# Autodesk Inventor assembly: toe_joint
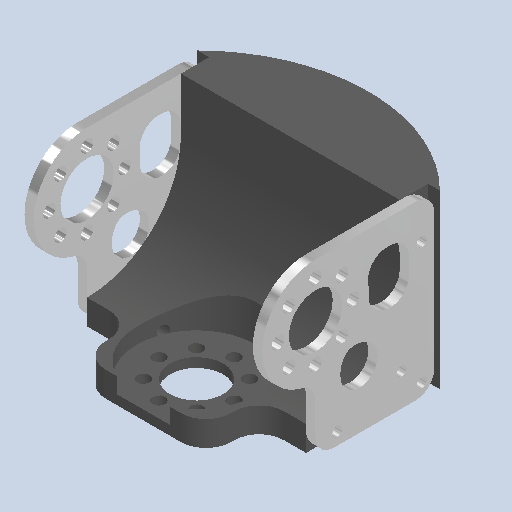
[picture p0: Inventor's stored thumbnail of the model, 512x512]
Saved by Autodesk Inventor 2024.1 (Build 281209000, 209)
## iProperties
Created: 2024-02-11
Part Number: toe_joint
Document SubType Name: Assembly
Designer: hibik
Author: hibik
## Documents named in this file (3)
- C:\Users\hibik\Desktop\ロボメカ\HR\2024.02.11 Rl\02.11 ProtType\toe_joint.iam
- C:\Users\hibik\Desktop\ロボメカ\HR\2024.02.11 Rl\02.11 ProtType\toe_joint_middle.ipt
- C:\Users\hibik\Desktop\ロボメカ\HR\2024.02.11 Rl\02.11 ProtType\toe_joint.ipt
## Components (3 placed, 2 different names)
1. toe_joint_middle:1 — メイト:1, メイト:2, フラッシュ:1, フラッシュ:2, フラッシュ:3, フラッシュ:4
2. toe_joint:1 — メイト:2, フラッシュ:1, フラッシュ:4
3. toe_joint:2 — メイト:1, フラッシュ:2, フラッシュ:3
## Relationships (6: Flush 4, Mate 2)
- メイト:1 [Mate]: toe_joint_middle:1 ↔ toe_joint:2
- メイト:2 [Mate]: toe_joint_middle:1 ↔ toe_joint:1
- フラッシュ:1 [Flush]: toe_joint_middle:1 ↔ toe_joint:1
- フラッシュ:2 [Flush]: toe_joint_middle:1 ↔ toe_joint:2
- フラッシュ:3 [Flush]: toe_joint_middle:1 ↔ toe_joint:2
- フラッシュ:4 [Flush]: toe_joint_middle:1 ↔ toe_joint:1
